# Autodesk Inventor assembly: gripper_and_camera_holder_
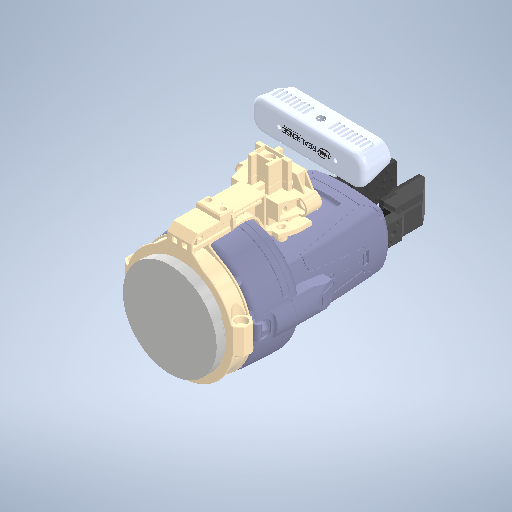
[picture p0: Inventor's stored thumbnail of the model, 512x512]
Saved by Autodesk Inventor 2025 (Build 290162010, 162A)
## iProperties
Created: 2024-08-06
Part Number: gripper_and_camera_holder_
Document SubType Name: Assembly
Designer: caubeeluck
Author: caubeeluck
## Documents named in this file (4)
- D:\Projects\Archived\Misc\github\autoclean\AutoClean\cad_files\gripper_and_camera_holder_assembly\gripper_and_camera_holder_.iam
- D:\Projects\Archived\Misc\github\autoclean\AutoClean\cad_files\gripper\final_models\gripper_assembly_open\schunk_with_gripper_fingers.iam
- D:\Projects\Archived\Misc\github\autoclean\AutoClean\cad_files\camera_holder\final_assembly_camera_holder_filleted.iam
- D:\Projects\Archived\Misc\github\autoclean\AutoClean\cad_files\depth_camera\RealSense_D435.ipt
## Components (3 placed, 3 different names)
1. schunk_with_gripper_fingers:1 [sub-assembly] — Mate:4
2. final_assembly_camera_holder_filleted:1 [sub-assembly] — Mate:2, Mate:3, Mate:4
3. RealSense_D435:1 — Mate:2, Mate:3
## Relationships (3: Mate 3)
- Mate:2: final_assembly_camera_holder_filleted:1 ↔ RealSense_D435:1
- Mate:3: final_assembly_camera_holder_filleted:1 ↔ RealSense_D435:1
- Mate:4: schunk_with_gripper_fingers:1 ↔ final_assembly_camera_holder_filleted:1
